# Autodesk Inventor assembly: Assembly1
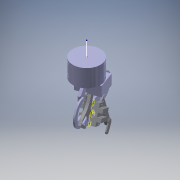
[picture p0: Inventor's stored thumbnail of the model, 180x180]
Saved by Autodesk Inventor 2018 (Build 220112000, 112)
## iProperties
Created: 2018-06-01
Part Number: Assembly1
Document SubType Name: Assembly
Designer: vigus
Author: vigus
## Documents named in this file (12)
- C:\Users\vigus\Documents\gihug\hecatonquiros\cad_models\accesories\muñeca\Assembly1.iam
- C:\Users\vigus\Documents\dji f550\muneca_rodamientos.ipt
- C:\Users\vigus\Documents\dji f550\muneca_rodamientos_1.ipt
- C:\Users\vigus\Documents\dji f550\muneca_rodamiento_2.ipt
- C:\Users\vigus\Documents\dji f550\muneca_rodamiento_3.ipt
- C:\Users\vigus\Documents\dji f550\motor.ipt
- C:\Users\vigus\Documents\gihug\hecatonquiros\cad_models\arm_4_dof\serial_model\microservo_FT.ipt
- C:\Users\vigus\Documents\gihug\hecatonquiros\cad_models\accesories\gripper\barra_1.ipt
- C:\Users\vigus\Documents\gihug\hecatonquiros\cad_models\accesories\gripper\barra_triangulo.ipt
- C:\Users\vigus\Documents\gihug\hecatonquiros\cad_models\accesories\gripper\garra_pilar_3.ipt
- C:\Users\vigus\Documents\gihug\hecatonquiros\cad_models\tools\gripper\serial_model_0dof\gripper.ipt
- C:\Users\vigus\Documents\gihug\hecatonquiros\cad_models\tools\gripper\serial_model_0dof\ScrewActuatorGripperCenter.ipt
## Components (15 placed, 11 different names)
1. muneca_rodamientos:1 — Mate:1, Mate:2, Mate:3, Mate:4
2. muneca_rodamientos_1:1 — Mate:1, Mate:2, Mate:5, Mate:6, Mate:7
3. muneca_rodamiento_2:1 — Mate:3, Mate:4, Mate:13
4. muneca_rodamiento_3:1 — Mate:5, Mate:6, Mate:7, Mate:8, Mate:9, Mate:10, Mate:11, Mate:12, Mate:14, Mate:15, Mate:16, Mate:17, Mate:21, Mate:22, Mate:23, Mate:24
5. motor:1 — Mate:8, Mate:9, Mate:10, Mate:11
6. microservo_FT:1 — Mate:12, Mate:13
7. barra_1:1 — Mate:21, Mate:22, Mate:25, Mate:26
8. barra_1:2 — Mate:14, Mate:15, Mate:19, Mate:20
9. barra_triangulo:1 — Mate:25, Mate:26, Mate:32, Mate:33
10. barra_triangulo:2 — Mate:19, Mate:20, Mate:29, Mate:34
11. garra_pilar_3:1 — Mate:16, Mate:17, Mate:27, Mate:28
12. garra_pilar_3:2 — Mate:23, Mate:24, Mate:30, Mate:31
13. gripper:1 — Mate:27, Mate:28, Mate:29
14. gripper:2 — Mate:30, Mate:31, Mate:32
15. ScrewActuatorGripperCenter:1 — Mate:33, Mate:34
## Relationships (33: Mate 33)
- Mate:1: muneca_rodamientos:1 ↔ muneca_rodamientos_1:1
- Mate:2: muneca_rodamientos:1 ↔ muneca_rodamientos_1:1
- Mate:3: muneca_rodamientos:1 ↔ muneca_rodamiento_2:1
- Mate:4: muneca_rodamientos:1 ↔ muneca_rodamiento_2:1
- Mate:5: muneca_rodamientos_1:1 ↔ muneca_rodamiento_3:1
- Mate:6: muneca_rodamientos_1:1 ↔ muneca_rodamiento_3:1
- Mate:7: muneca_rodamientos_1:1 ↔ muneca_rodamiento_3:1
- Mate:8: muneca_rodamiento_3:1 ↔ motor:1
- Mate:9: muneca_rodamiento_3:1 ↔ motor:1
- Mate:10: muneca_rodamiento_3:1 ↔ motor:1
- Mate:11: muneca_rodamiento_3:1 ↔ motor:1
- Mate:12: muneca_rodamiento_3:1 ↔ microservo_FT:1
- Mate:13: muneca_rodamiento_2:1 ↔ microservo_FT:1
- Mate:14: muneca_rodamiento_3:1 ↔ barra_1:2
- Mate:15: muneca_rodamiento_3:1 ↔ barra_1:2
- Mate:16: muneca_rodamiento_3:1 ↔ garra_pilar_3:1
- Mate:17: muneca_rodamiento_3:1 ↔ garra_pilar_3:1
- Mate:19: barra_1:2 ↔ barra_triangulo:2
- Mate:20: barra_1:2 ↔ barra_triangulo:2
- Mate:21: muneca_rodamiento_3:1 ↔ barra_1:1
- Mate:22: muneca_rodamiento_3:1 ↔ barra_1:1
- Mate:23: muneca_rodamiento_3:1 ↔ garra_pilar_3:2
- Mate:24: muneca_rodamiento_3:1 ↔ garra_pilar_3:2
- Mate:25: barra_1:1 ↔ barra_triangulo:1
- Mate:26: barra_1:1 ↔ barra_triangulo:1
- Mate:27: garra_pilar_3:1 ↔ gripper:1
- Mate:28: garra_pilar_3:1 ↔ gripper:1
- Mate:29: barra_triangulo:2 ↔ gripper:1
- Mate:30: garra_pilar_3:2 ↔ gripper:2
- Mate:31: garra_pilar_3:2 ↔ gripper:2
- Mate:32: barra_triangulo:1 ↔ gripper:2
- Mate:33: barra_triangulo:1 ↔ ScrewActuatorGripperCenter:1
- Mate:34: barra_triangulo:2 ↔ ScrewActuatorGripperCenter:1
